# Autodesk Inventor assembly: RFID_Machine_Access_Node_v1
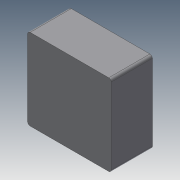
[picture p0: Inventor's stored thumbnail of the model, 180x180]
Saved by Autodesk Inventor 2014 SP1 (Build 180222100, 222)
## iProperties
Created: 2015-04-01
Part Number: RFID_Machine_Access_Node_v1
Document SubType Name: Assembly
Designer: tom
Author: tom
## Documents named in this file (5)
- C:\Users\tom\Documents\Work\Tinkermill\RFID Machine Access Node\Inventor\RFID_Machine_Access_Node_v1.iam
- C:\Users\tom\Documents\Work\Tinkermill\RFID Machine Access Node\Inventor\Part1.ipt
- C:\Users\tom\Documents\Work\Tinkermill\RFID Machine Access Node\Inventor\LCD.ipt
- C:\Users\tom\Documents\Work\Tinkermill\RFID Machine Access Node\Inventor\Part3.ipt
- C:\Users\tom\Documents\Work\Tinkermill\RFID Machine Access Node\Inventor\Part4.ipt
## Components (4 placed, 4 different names)
1. Part1:1 — Flush:1, Flush:2, Mate:1, Mate:2, Flush:3, Mate:5, Flush:7, Mate:6, Flush:8
2. LCD:1 — Flush:2, Mate:1, Mate:2, Mate:3, Angle:1
3. Part3:1 — Flush:1
4. Part4:1 — Mate:5, Flush:7, Mate:6, Mate:7, Angle:2
## Relationships (13: Mate 6, Flush 5, Angle 2)
- Flush:1: Part1:1 ↔ Part3:1
- Flush:2 (2 mm): Part1:1 ↔ LCD:1
- Mate:1 (2.8625 mm): Part1:1 ↔ LCD:1
- Mate:2 (2.8625 mm): Part1:1 ↔ LCD:1
- Mate:3: LCD:1
- Angle:1 (0 deg): LCD:1
- Flush:3: Part1:1
- Mate:5 (2.8625 mm): Part1:1 ↔ Part4:1
- Flush:7 (20 mm): Part1:1 ↔ Part4:1
- Mate:6 (2.8625 mm): Part1:1 ↔ Part4:1
- Mate:7: Part4:1
- Angle:2 (0 deg): Part4:1
- Flush:8: Part1:1
